# Autodesk Inventor assembly: Dragon Hotend ST-SF&HF
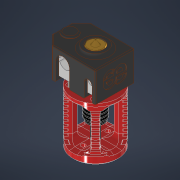
[picture p0: Inventor's stored thumbnail of the model, 180x180]
Saved by Autodesk Inventor 2022.2 (Build 262287010, 287A)
## iProperties
Created: 2022-01-01
Part Number: Dragon Hotend ST-SF&HF
Document SubType Name: Assembly
Designer: sleib
Sending System: Autodesk Translation Framework v10.10.0.1391
Preprocessor: ST-DEVELOPER v18.1
Title: /Users/tobiasmurday/Downloads/Dragon Hotend ST-SF&HF.step
## Documents named in this file (7)
- C:\Users\sleib\Projekte\Voron-2\CAD\Inventor\Dragon Hotend\Dragon Hotend.iam
- C:\Users\sleib\Projekte\Voron-2\CAD\Inventor\Dragon Hotend\heatsink.ipt
- C:\Users\sleib\Projekte\Voron-2\CAD\Inventor\Dragon Hotend\block standoffs.ipt
- Block Standoffs.ipt
- C:\Users\sleib\Projekte\Voron-2\CAD\Inventor\Dragon Hotend\block.ipt
- Block.ipt
- C:\Users\sleib\Projekte\Voron-2\CAD\Inventor\Dragon Hotend\V6 Nozzle.ipt
## Components (4 placed, 4 different names)
1. Heatsink:1 — Passend:3, Passend:4, Passend:5
2. Block Standoffs:1 — Passend:3, Passend:4, Passend:5, Passend:6, Passend:7, Passend:8
3. Block:1 — Passend:6, Passend:7, Passend:8, Passend:9, Passend:10
4. V6 Nozzle:1 — Passend:9, Passend:10
## Relationships (8: Mate 8)
- Passend:3 [Mate]: Heatsink:1 ↔ Block Standoffs:1
- Passend:4 [Mate]: Heatsink:1 ↔ Block Standoffs:1
- Passend:5 [Mate]: Heatsink:1 ↔ Block Standoffs:1
- Passend:6 [Mate]: Block Standoffs:1 ↔ Block:1
- Passend:7 [Mate]: Block Standoffs:1 ↔ Block:1
- Passend:8 [Mate]: Block Standoffs:1 ↔ Block:1
- Passend:9 [Mate]: Block:1 ↔ V6 Nozzle:1
- Passend:10 [Mate]: Block:1 ↔ V6 Nozzle:1
